# Autodesk Inventor assembly: Assembly Box
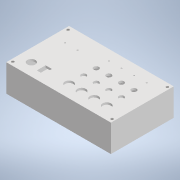
[picture p0: Inventor's stored thumbnail of the model, 180x180]
Saved by Autodesk Inventor 2022 (Build 260153000, 153)
## iProperties
Created: 2021-07-04
Part Number: Assembly Box
Document SubType Name: Assembly
Designer: Matthijs
Author: Matthijs
## Documents named in this file (5)
- C:\Users\MJAC\Desktop\3D-Box\Assembly Box.iam
- C:\Users\MJAC\Desktop\3D-Box\Box Top.ipt
- C:\Users\MJAC\Desktop\3D-Box\Box.ipt
- C:\Users\Matthijs\Documents\Inventor\Content Center Files\R2022\en-US\ISO 4762(2)\ISO 4762 - M3 x 10ISO.ipt
- C:\Users\MJAC\Documents\Inventor\Content Center Files\R2022\en-US\ISO 4762(2)\ISO 4762 - M3 x 16ISO.ipt
## Components (10 placed, 4 different names)
1. Box Top:1 — Flush:1, Flush:2, Mate:1, Insert:1, Insert:2, Insert:3, Insert:4, Flush:3
2. Box:1 — Flush:1, Flush:2, Mate:1, Flush:3
3. ISO 4762 M3 x 10:1
4. ISO 4762 M3 x 10:2
5. ISO 4762 M3 x 10:3
6. ISO 4762 M3 x 10:4
7. ISO 4762 M3 x 16:1 — Insert:1
8. ISO 4762 M3 x 16:2 — Insert:2
9. ISO 4762 M3 x 16:3 — Insert:3
10. ISO 4762 M3 x 16:4 — Insert:4
## Relationships (8: Insert 4, Flush 3, Mate 1)
- Flush:1: Box Top:1 ↔ Box:1
- Flush:2: Box Top:1 ↔ Box:1
- Mate:1: Box Top:1 ↔ Box:1
- Insert:1: Box Top:1 ↔ ISO 4762 M3 x 16:1
- Insert:2: Box Top:1 ↔ ISO 4762 M3 x 16:2
- Insert:3: Box Top:1 ↔ ISO 4762 M3 x 16:3
- Insert:4: Box Top:1 ↔ ISO 4762 M3 x 16:4
- Flush:3: Box Top:1 ↔ Box:1
